# Autodesk Inventor assembly: Connecteur jst 4 broches
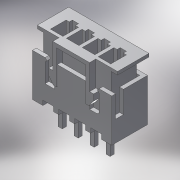
[picture p0: Inventor's stored thumbnail of the model, 180x180]
Saved by Autodesk Inventor 2017 (Build 210142000, 142)
## iProperties
Part Number: Connecteur jst 4 broches
Material: Générique
Document SubType Name: Assembly
Designer: Adrien MARY
Author: Adrien MARY
## Documents named in this file (10)
- W:\Professionnel\Conception FABLAB\1410-LaserShow\1410-04 Connecteur_JST\Connecteur_JST.iam
- W:\Professionnel\Conception FABLAB\1410-LaserShow\1410-04 Connecteur_JST\Connecteur_jst_femelle.ipt
- W:\Professionnel\Conception FABLAB\1410-LaserShow\1410-04 Connecteur_JST\Connecteur_jst_male.ipt
- W:\Professionnel\Conception FABLAB\1410-LaserShow\1410-04 Connecteur_JST\Connecteur_jst_femelle\Connecteur jst 4 broches femelle.ipt
- W:\Professionnel\Conception FABLAB\1410-LaserShow\1410-04 Connecteur_JST\Connecteur_jst_male\Connecteur JST 4 Broches Male.ipt
- Connecteur jst 2 broches.iam
- Connecteur jst 3 broches.iam
- Connecteur jst 4 broches.iam
- Connecteur jst 5 broches.iam
- Connecteur jst 6 broches.iam
## Components (2 placed, 2 different names)
1. Connecteur jst 4 broches femelle:1 — Affleurement:1, Affleurement:2, Affleurement:3, Placage:1
2. Connecteur JST 4 Broches Male:1 — Placage:1, Placage:2, Placage:3
## Relationships (6: Flush 3, Mate 3)
- Affleurement:1 [Flush]: Connecteur jst 4 broches femelle:1
- Affleurement:2 [Flush]: Connecteur jst 4 broches femelle:1
- Affleurement:3 [Flush]: Connecteur jst 4 broches femelle:1
- Placage:1 [Mate]: Connecteur jst 4 broches femelle:1 ↔ Connecteur JST 4 Broches Male:1
- Placage:2 [Mate]: Connecteur JST 4 Broches Male:1
- Placage:3 [Mate]: Connecteur JST 4 Broches Male:1
